# Autodesk Inventor assembly: frame
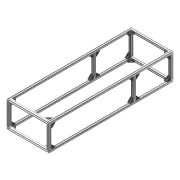
[picture p0: Inventor's stored thumbnail of the model, 180x180]
Saved by Autodesk Inventor 2017 (Build 210142000, 142)
## iProperties
Created: 2017-03-01
Part Number: frame
Document SubType Name: Assembly
Designer: sawaiz
Author: sawaiz
## Documents named in this file (6)
- C:\Users\sawaiz\oneDrive\projects\sPhenixTileTestStand\frame\frame.iam
- C:\Users\sawaiz\oneDrive\projects\sPhenixTileTestStand\frame\hfs5-2020Width.ipt
- C:\Users\sawaiz\oneDrive\projects\sPhenixTileTestStand\frame\leftSide.iam
- C:\Users\sawaiz\oneDrive\projects\sPhenixTileTestStand\frame\rightSide.iam
- C:\Users\sawaiz\oneDrive\projects\sPhenixTileTestStand\hardware\angleBracket.iam
- C:\Users\sawaiz\oneDrive\projects\sPhenixTileTestStand\sPhenixTileTestStand.xlsx
## Components (14 placed, 4 different names)
1. leftSide:1 [sub-assembly] — Flush:1, Flush:2, Symmetry:1, Symmetry:2, Symmetry:3, Flush:3, Flush:4, Mate:2, Angle:4, Flush:12, Mate:4, Mate:10, Mate:11, Mate:13
2. rightSide:1 [sub-assembly] — Flush:1, Flush:2, Symmetry:1, Symmetry:2, Symmetry:3, Mate:1, Mate:5, Mate:7, Mate:12, Mate:14
3. angleBracket:1 [sub-assembly] — Angle:7, Angle:8, Flush:5, Flush:9, Flush:10, Mate:7, Mate:8
4. angleBracket:2 [sub-assembly] — Angle:1, Flush:8, Flush:10, Flush:11, Mate:5, Mate:6
5. angleBracket:3 [sub-assembly] — Angle:2, Angle:3, Flush:7, Flush:15, Flush:16, Mate:11
6. angleBracket:4 [sub-assembly] — Angle:6, Angle:7, Flush:6, Flush:9, Mate:9, Mate:10
7. angleBracket:5 [sub-assembly] — Angle:5, Angle:6, Flush:6, Flush:13, Mate:13
8. angleBracket:6 [sub-assembly] — Angle:8, Flush:5, Flush:13, Flush:14, Mate:14
9. angleBracket:7 [sub-assembly] — Angle:1, Angle:2, Flush:8, Flush:14, Flush:15, Mate:12
10. angleBracket:8 [sub-assembly] — Angle:3, Angle:4, Angle:5, Flush:7, Flush:11, Flush:12, Mate:3, Mate:4
11. hfs5-2020Width:1 — Flush:3, Flush:4, Mate:1, Mate:2, Mate:8, Mate:9
12. hfs5-2020Width:2
13. hfs5-2020Width:3 — Mate:3, Mate:6
14. hfs5-2020Width:4 — Flush:16
## Component patterns: (4 elements, first: hfs5-2020Width:1)
## Relationships (41: Flush 16, Mate 14, Angle 8, Symmetry 3)
- Flush:1: leftSide:1 ↔ rightSide:1
- Flush:2: leftSide:1 ↔ rightSide:1
- Symmetry:1: leftSide:1 ↔ rightSide:1
- Symmetry:2: leftSide:1 ↔ rightSide:1
- Symmetry:3: leftSide:1 ↔ rightSide:1
- Flush:3: leftSide:1 ↔ hfs5-2020Width:1
- Flush:4: leftSide:1 ↔ hfs5-2020Width:1
- Mate:1: rightSide:1 ↔ hfs5-2020Width:1
- Mate:2: leftSide:1 ↔ hfs5-2020Width:1
- Angle:1 (0 deg): angleBracket:2 ↔ angleBracket:7
- Angle:2 (0 deg): angleBracket:3 ↔ angleBracket:7
- Angle:3 (0 deg): angleBracket:3 ↔ angleBracket:8
- Angle:4 (0 deg): leftSide:1 ↔ angleBracket:8
- Angle:5 (0 deg): angleBracket:5 ↔ angleBracket:8
- Angle:6 (0 deg): angleBracket:4 ↔ angleBracket:5
- Angle:7 (0 deg): angleBracket:1 ↔ angleBracket:4
- Angle:8 (0 deg): angleBracket:1 ↔ angleBracket:6
- Flush:5: angleBracket:1 ↔ angleBracket:6
- Flush:6: angleBracket:4 ↔ angleBracket:5
- Flush:7: angleBracket:3 ↔ angleBracket:8
- Flush:8: angleBracket:2 ↔ angleBracket:7
- Flush:9: angleBracket:1 ↔ angleBracket:4
- Flush:10: angleBracket:1 ↔ angleBracket:2
- Flush:11: angleBracket:2 ↔ angleBracket:8
- Flush:12: leftSide:1 ↔ angleBracket:8
- Mate:3: angleBracket:8 ↔ hfs5-2020Width:3
- Mate:4: leftSide:1 ↔ angleBracket:8
- Mate:5: rightSide:1 ↔ angleBracket:2
- Mate:6: angleBracket:2 ↔ hfs5-2020Width:3
- Mate:7: rightSide:1 ↔ angleBracket:1
- Mate:8: angleBracket:1 ↔ hfs5-2020Width:1
- Mate:9: angleBracket:4 ↔ hfs5-2020Width:1
- Mate:10: leftSide:1 ↔ angleBracket:4
- Flush:13: angleBracket:5 ↔ angleBracket:6
- Flush:14: angleBracket:6 ↔ angleBracket:7
- Flush:15: angleBracket:3 ↔ angleBracket:7
- Flush:16: angleBracket:3 ↔ hfs5-2020Width:4
- Mate:11: leftSide:1 ↔ angleBracket:3
- Mate:12: rightSide:1 ↔ angleBracket:7
- Mate:13: leftSide:1 ↔ angleBracket:5
- Mate:14: rightSide:1 ↔ angleBracket:6
## Named parameters: plateWidth = 300 mm, plateDepth = 1000 mm, supportPlateThickness = 6.35 mm, supportPlateWidth = 50 mm, supportPlateFillet = 10 mm, separation = 35 mm, numPanels = 5, centerVerticalRatio = 0.3
